# Autodesk Inventor assembly: Final Assembly
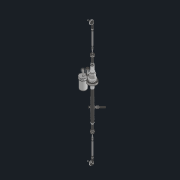
[picture p0: Inventor's stored thumbnail of the model, 180x180]
Saved by Autodesk Inventor 2021 (Build 250183000, 183)
## iProperties
Created: 2020-10-21
Part Number: Final Assembly
Document SubType Name: Assembly
Designer: Tang Kang Ning
Mass: 19906 g
Surface Area: 15225.4 cm^2
Volume: 4263.88 cm^3
Density: 4.66852 g/cm^3
Author: Tang Kang Ning
## Documents named in this file (41)
- C:\Users\teuge\OneDrive - Curtin University of Technology Australia\Y4S2\DFM\Group Project\CAD\Final Assembly.iam
- C:\Users\teuge\OneDrive - Curtin University of Technology Australia\Y4S2\DFM\Group Project\CAD\Parts\Steering Rack.ipt
- C:\Users\teuge\OneDrive - Curtin University of Technology Australia\Y4S2\DFM\Group Project\CAD\Parts\Shell Body.ipt
- C:\Users\teuge\OneDrive - Curtin University of Technology Australia\Y4S2\DFM\Group Project\CAD\Parts\Assemblies\Bearing2.iam
- C:\Users\teuge\OneDrive - Curtin University of Technology Australia\Y4S2\DFM\Group Project\CAD\Parts\Steering Gear.ipt
- C:\Users\teuge\OneDrive - Curtin University of Technology Australia\Y4S2\DFM\Group Project\CAD\Parts\Steering Shaft.ipt
- C:\Users\teuge\OneDrive - Curtin University of Technology Australia\Y4S2\DFM\Group Project\CAD\Parts\Assemblies\Bearing1.iam
- C:\Users\teuge\OneDrive - Curtin University of Technology Australia\Y4S2\DFM\Group Project\CAD\Parts\Assemblies\Motor Assembly.iam
- C:\Users\teuge\OneDrive - Curtin University of Technology Australia\Y4S2\DFM\Group Project\CAD\Parts\Gear Key.ipt
- C:\Users\teuge\OneDrive - Curtin University of Technology Australia\Y4S2\DFM\Group Project\CAD\Parts\Gears\Gear.ipt
- C:\Users\teuge\OneDrive - Curtin University of Technology Australia\Y4S2\DFM\Group Project\CAD\Parts\Intermediate Gear Pin.ipt
- C:\Users\teuge\OneDrive - Curtin University of Technology Australia\Y4S2\DFM\Group Project\CAD\Parts\Assemblies\Bearing7.iam
- C:\Users\teuge\OneDrive - Curtin University of Technology Australia\Y4S2\DFM\Group Project\CAD\Parts\Intermediate Key.ipt
- C:\Users\teuge\OneDrive - Curtin University of Technology Australia\Y4S2\DFM\Group Project\CAD\Parts\Gears\Intermediate.ipt
- C:\Users\teuge\OneDrive - Curtin University of Technology Australia\Y4S2\DFM\Group Project\CAD\Parts\Pinion.ipt
- C:\Users\teuge\OneDrive - Curtin University of Technology Australia\Y4S2\DFM\Group Project\CAD\Parts\PinionMotor Key.ipt
- C:\Users\teuge\OneDrive - Curtin University of Technology Australia\Y4S2\DFM\Group Project\CAD\Parts\Shell Cap.ipt
- C:\Users\teuge\OneDrive - Curtin University of Technology Australia\Y4S2\DFM\Group Project\CAD\Parts\Assemblies\Tie Rod Assembly.iam
- C:\Users\teuge\OneDrive - Curtin University of Technology Australia\Y4S2\DFM\Group Project\CAD\Parts\Screws\ISO 4762 - M6 x 40ISO.ipt
- C:\Users\teuge\OneDrive - Curtin University of Technology Australia\Y4S2\DFM\Group Project\CAD\Parts\Screws\ISO 4762 - M8 x 20ISO.ipt
- C:\Users\teuge\OneDrive - Curtin University of Technology Australia\Y4S2\DFM\Group Project\CAD\Parts\Boot front.ipt
- C:\Users\teuge\OneDrive - Curtin University of Technology Australia\Y4S2\DFM\Group Project\CAD\Parts\Boot Back.ipt
- C:\Users\teuge\OneDrive - Curtin University of Technology Australia\Y4S2\DFM\Group Project\CAD\Final Assembly\Design Accelerator\Involute Spline Connection1.iam
- C:\Users\teuge\OneDrive - Curtin University of Technology Australia\Y4S2\DFM\Group Project\CAD\Final Assembly\Design Accelerator\Bearing1.iam
- C:\Users\teuge\OneDrive - Curtin University of Technology Australia\Y4S2\DFM\Group Project\CAD\Parts\Nut Fastener.ipt
- C:\Users\teuge\OneDrive - Curtin University of Technology Australia\Y4S2\DFM\Group Project\CAD\Parts\Out Tie Rod Joint Cap.ipt
- C:\Users\teuge\OneDrive - Curtin University of Technology Australia\Y4S2\DFM\Group Project\CAD\Parts\Outer Tie Rod Ball.ipt
- C:\Users\teuge\OneDrive - Curtin University of Technology Australia\Y4S2\DFM\Group Project\CAD\Parts\Outer Tie Rod.ipt
- C:\Users\teuge\OneDrive - Curtin University of Technology Australia\Y4S2\DFM\Group Project\CAD\Master\Inner Ball Joint (Body).ipt
- C:\Users\teuge\OneDrive - Curtin University of Technology Australia\Y4S2\DFM\Group Project\CAD\Master\Inner Ball Joint (Cap).ipt
- C:\Users\teuge\OneDrive - Curtin University of Technology Australia\Y4S2\DFM\Group Project\CAD\Master\Tie Rod.ipt
- C:\Users\teuge\OneDrive - Curtin University of Technology Australia\Y4S2\DFM\Group Project\CAD\Master\Ball Screw Nut 1.0.ipt
- C:\Users\teuge\OneDrive - Curtin University of Technology Australia\Y4S2\DFM\Group Project\CAD\Parts\Ball Screw Balls.ipt
- C:\Users\teuge\OneDrive - Curtin University of Technology Australia\Y4S2\DFM\Group Project\CAD\Master\Front Returd Mech.ipt
- C:\Users\teuge\OneDrive - Curtin University of Technology Australia\Y4S2\DFM\Group Project\CAD\Master\BallScrewNut Cap.ipt
- C:\Users\teuge\OneDrive - Curtin University of Technology Australia\Y4S2\DFM\Group Project\CAD\Final Assembly\AIP\FEA\dejyt38kg.fins
- C:\Users\teuge\OneDrive - Curtin University of Technology Australia\Y4S2\DFM\Group Project\CAD\Final Assembly\AIP\FEA\dejyt38kg.fsat
- C:\Users\teuge\OneDrive - Curtin University of Technology Australia\Y4S2\DFM\Group Project\CAD\Final Assembly\AIP\FEA\dejyt38kg.ftes
- C:\Users\teuge\OneDrive - Curtin University of Technology Australia\Y4S2\DFM\Group Project\CAD\Final Assembly\AIP\FEA\dejyt38kg.fwiz
- C:\Users\teuge\OneDrive - Curtin University of Technology Australia\Y4S2\DFM\Group Project\CAD\Final Assembly\AIP\FEA\dekbs9e9s.fmsh
- C:\Users\teuge\OneDrive - Curtin University of Technology Australia\Y4S2\DFM\Group Project\CAD\Final Assembly\AIP\FEA\dekbs9e9t.fres
## Components (51 placed, 31 different names)
1. Steering Rack:1 — Mate:1, Mate:2, Mate:3, Mate:4, Mate:5, Position Adjust, Mate:45, Mate:49, Mate:50, Flush:6, Mate:85, Mate:87, Mate:127, Mate:133, Mate:134
2. Bearing:1 [sub-assembly] — Mate:48
3. Bearing:2 [sub-assembly] — Mate:28
4. Steering Gear:1 — Mate:11, Mate:14
5. Steering Shaft:1 — Mate:11, Mate:12, Flush:1, Mate:13, Mate:14, Position Adjust, Mate:74, Mate:75
6. Bearing:3 [sub-assembly] — Mate:12, Flush:1, Mate:15
7. Motor Assembly:1 [sub-assembly] — Mate:17, Mate:18, Mate:19, Mate:20, Mate:39, Mate:40, Mate:42, Mate:60, Mate:61, Mate:62, Mate:63, Mate:64, Mate:132
8. Gear Key:1 — Mate:79, Mate:125, Mate:126, Mate:129
9. Gear:1 — Flush:4, Mate:79, Mate:128
10. Intermediate Gear Pin:1 — Mate:29, Mate:30, Mate:32, Flush:2, Mate:33, Flush:3, Mate:34, Mate:131
11. Bearing:4 [sub-assembly] — Mate:32, Flush:2, Mate:37, Mate:38
12. Intermediate Key:1 — Mate:29, Mate:30, Mate:35, Mate:36, Mate:131
13. Bearing:5 [sub-assembly] — Mate:33, Flush:3, Mate:130
14. Intermediate:1 — Mate:34, Mate:35, Mate:36, Flush:4, Flush:5
15. Pinion:1 — Mate:42, Mate:43, Mate:44, Flush:5
16. PinionMotor Key:1 — Mate:39, Mate:40, Mate:43, Mate:44, Mate:132
17. Boot front:1 — Mate:70, Mate:71
18. Boot Back:1 — Mate:72, Mate:73
19. Involute Spline Connection:1 [sub-assembly]
20. Bearing:6 [sub-assembly] — Mate:74, Mate:75
21. Out Tie Rod Joint Cap:1 — Mate:102, Mate:103
22. Outer Tie Rod Ball:1 — Mate:82, Mate:101, Mate:112
23. Outer Tie Rod:1 — Mate:82, Mate:101, Mate:102, Mate:103, Mate:104, Mate:110
24. Out Tie Rod Joint Cap:2 — Mate:84, Mate:99
25. Outer Tie Rod Ball:2 — Mate:83, Mate:84, Mate:100, Mate:111
26. Outer Tie Rod:2 — Mate:83, Mate:98, Mate:99, Mate:100, Mate:107
27. Inner Ball Joint (Body):1 — Mate:85, Mate:93, Mate:94, Mate:134
28. Inner Ball Joint (Cap):1 — Mate:93, Mate:94, Mate:95, Mate:97
29. Tie Rod:1 — Mate:95, Mate:97, Mate:98, Mate:105, Mate:106
30. Inner Ball Joint (Body):2 — Mate:87, Mate:90, Mate:91, Mate:92, Mate:133
31. Inner Ball Joint (Cap):2 — Mate:90, Mate:91, Mate:96
32. Tie Rod:2 — Mate:92, Mate:96, Mate:104, Mate:108, Mate:109
33. Nut Fastener:1 — Mate:108, Mate:109, Mate:110
34. Nut Fastener:2 — Mate:105, Mate:106, Mate:107
35. Ball Screw Nut 1.0:1 — Mate:113, Mate:114, Mate:115, Mate:116, Mate:117, Mate:118, Mate:119, Mate:120, Mate:121, Mate:122, Mate:123, Mate:124, Mate:125, Mate:126, Mate:127, Mate:128, Mate:129
36. Ball Screw Balls:1 — Mate:113, Mate:114
37. Front Returd Mech:1 — Mate:115, Mate:116, Mate:117
38. Front Returd Mech:2 — Mate:118, Mate:119, Mate:120
39. BallScrewNut Cap:1 — Mate:122, Mate:123
40. BallScrewNut Cap:2 — Mate:121, Mate:124
41. ISO 4762 - M6 x 40ISO:1 — Mate:60, Mate:63
42. ISO 4762 - M8 x 20ISO:1 — Mate:57, Mate:65
43. ISO 4762 - M6 x 40ISO:2 — Mate:61, Mate:64
44. ISO 4762 - M8 x 20ISO:2 — Mate:56, Mate:66
45. ISO 4762 - M6 x 40ISO:3 — Mate:59, Mate:62
46. ISO 4762 - M8 x 20ISO:3 — Mate:58, Mate:67
47. ISO 4762 - M8 x 20ISO:4 — Mate:55, Mate:68
48. Shell Body:1 — Mate:1, Mate:2, Mate:13, Mate:15, Mate:17, Mate:18, Mate:19, Mate:20, Mate:28, Mate:37, Mate:38, Mate:46, Mate:47, Mate:56, Mate:59, Mate:72, Mate:73
49. Shell Cap:1 — Mate:45, Mate:46, Mate:47, Mate:48, Mate:55, Mate:57, Mate:58, Mate:65, Mate:66, Mate:67, Mate:68, Mate:71, Mate:130
50. Tie Rod Assembly:1 [sub-assembly] — Mate:50, Mate:54, Mate:70
51. Tie Rod Assembly:2 [sub-assembly] — Mate:49, Mate:53
## Relationships (115: Mate 109, Flush 6)
- Mate:1: Steering Rack:1 ↔ Shell Body:1
- Mate:2: Steering Rack:1 ↔ Shell Body:1
- Mate:3: Steering Rack:1
- Mate:4: Steering Rack:1
- Mate:5: Steering Rack:1
- Mate:11: Steering Gear:1 ↔ Steering Shaft:1
- Mate:12: Steering Shaft:1 ↔ Bearing:3
- Flush:1: Steering Shaft:1 ↔ Bearing:3
- Mate:13: Steering Shaft:1 ↔ Shell Body:1
- Mate:14: Steering Gear:1 ↔ Steering Shaft:1
- Mate:15: Bearing:3 ↔ Shell Body:1
- Position Adjust [Mate] (-2.75 mm): Steering Rack:1 ↔ Steering Shaft:1
- Mate:17: Motor Assembly:1 ↔ Shell Body:1
- Mate:18: Motor Assembly:1 ↔ Shell Body:1
- Mate:19: Motor Assembly:1 ↔ Shell Body:1
- Mate:20: Motor Assembly:1 ↔ Shell Body:1
- Mate:28: Bearing:2 ↔ Shell Body:1
- Mate:29: Intermediate Gear Pin:1 ↔ Intermediate Key:1
- Mate:30: Intermediate Gear Pin:1 ↔ Intermediate Key:1
- Mate:32: Intermediate Gear Pin:1 ↔ Bearing:4
- Flush:2: Intermediate Gear Pin:1 ↔ Bearing:4
- Mate:33: Intermediate Gear Pin:1 ↔ Bearing:5
- Flush:3: Intermediate Gear Pin:1 ↔ Bearing:5
- Mate:34: Intermediate Gear Pin:1 ↔ Intermediate:1
- Mate:35: Intermediate Key:1 ↔ Intermediate:1
- Mate:36: Intermediate Key:1 ↔ Intermediate:1
- Mate:37: Bearing:4 ↔ Shell Body:1
- Mate:38: Bearing:4 ↔ Shell Body:1
- Flush:4: Gear:1 ↔ Intermediate:1
- Mate:39: Motor Assembly:1 ↔ PinionMotor Key:1
- Mate:40: Motor Assembly:1 ↔ PinionMotor Key:1
- Mate:42: Motor Assembly:1 ↔ Pinion:1
- Mate:43: Pinion:1 ↔ PinionMotor Key:1
- Mate:44: Pinion:1 ↔ PinionMotor Key:1
- Flush:5: Intermediate:1 ↔ Pinion:1
- Mate:45: Steering Rack:1 ↔ Shell Cap:1
- Mate:46: Shell Body:1 ↔ Shell Cap:1
- Mate:47: Shell Body:1 ↔ Shell Cap:1
- Mate:48: Bearing:1 ↔ Shell Cap:1
- Mate:49: Steering Rack:1 ↔ Tie Rod Assembly:2
- Mate:50: Steering Rack:1 ↔ Tie Rod Assembly:1
- Mate:53: Tie Rod Assembly:2
- Mate:54: Tie Rod Assembly:1
- Mate:55: ISO 4762 - M8 x 20ISO:4 ↔ Shell Cap:1
- Mate:56: ISO 4762 - M8 x 20ISO:2 ↔ Shell Body:1
- Mate:57: ISO 4762 - M8 x 20ISO:1 ↔ Shell Cap:1
- Mate:58: ISO 4762 - M8 x 20ISO:3 ↔ Shell Cap:1
- Mate:59: ISO 4762 - M6 x 40ISO:3 ↔ Shell Body:1
- Mate:60: Motor Assembly:1 ↔ ISO 4762 - M6 x 40ISO:1
- Mate:61: Motor Assembly:1 ↔ ISO 4762 - M6 x 40ISO:2
- Mate:62: Motor Assembly:1 ↔ ISO 4762 - M6 x 40ISO:3
- Mate:63: Motor Assembly:1 ↔ ISO 4762 - M6 x 40ISO:1
- Mate:64: Motor Assembly:1 ↔ ISO 4762 - M6 x 40ISO:2
- Mate:65: ISO 4762 - M8 x 20ISO:1 ↔ Shell Cap:1
- Mate:66: ISO 4762 - M8 x 20ISO:2 ↔ Shell Cap:1
- Mate:67: ISO 4762 - M8 x 20ISO:3 ↔ Shell Cap:1
- Mate:68: ISO 4762 - M8 x 20ISO:4 ↔ Shell Cap:1
- Flush:6: Steering Rack:1
- Mate:70: Boot front:1 ↔ Tie Rod Assembly:1
- Mate:71: Boot front:1 ↔ Shell Cap:1
- Mate:72: Boot Back:1 ↔ Shell Body:1
- Mate:73: Boot Back:1 ↔ Shell Body:1
- Mate:74: Steering Shaft:1 ↔ Bearing:6
- Mate:75: Steering Shaft:1 ↔ Bearing:6
- Mate:79: Gear Key:1 ↔ Gear:1
- Mate:82: Outer Tie Rod Ball:1 ↔ Outer Tie Rod:1
- Mate:83: Outer Tie Rod Ball:2 ↔ Outer Tie Rod:2
- Mate:84: Out Tie Rod Joint Cap:2 ↔ Outer Tie Rod Ball:2
- Mate:85: Steering Rack:1 ↔ Inner Ball Joint (Body):1
- Mate:87: Steering Rack:1 ↔ Inner Ball Joint (Body):2
- Mate:90: Inner Ball Joint (Body):2 ↔ Inner Ball Joint (Cap):2
- Mate:91: Inner Ball Joint (Body):2 ↔ Inner Ball Joint (Cap):2
- Mate:92: Inner Ball Joint (Body):2 ↔ Tie Rod:2
- Mate:93: Inner Ball Joint (Body):1 ↔ Inner Ball Joint (Cap):1
- Mate:94: Inner Ball Joint (Body):1 ↔ Inner Ball Joint (Cap):1
- Mate:95: Inner Ball Joint (Cap):1 ↔ Tie Rod:1
- Mate:96: Inner Ball Joint (Cap):2 ↔ Tie Rod:2
- Mate:97: Inner Ball Joint (Cap):1 ↔ Tie Rod:1
- Mate:98: Outer Tie Rod:2 ↔ Tie Rod:1
- Mate:99: Out Tie Rod Joint Cap:2 ↔ Outer Tie Rod:2
- Mate:100: Outer Tie Rod Ball:2 ↔ Outer Tie Rod:2
- Mate:101: Outer Tie Rod Ball:1 ↔ Outer Tie Rod:1
- Mate:102: Out Tie Rod Joint Cap:1 ↔ Outer Tie Rod:1
- Mate:103: Out Tie Rod Joint Cap:1 ↔ Outer Tie Rod:1
- Mate:104: Outer Tie Rod:1 ↔ Tie Rod:2
- Mate:105: Tie Rod:1 ↔ Nut Fastener:2
- Mate:106 (7.8 mm): Tie Rod:1 ↔ Nut Fastener:2
- Mate:107: Outer Tie Rod:2 ↔ Nut Fastener:2
- Mate:108: Tie Rod:2 ↔ Nut Fastener:1
- Mate:109 (7.8 mm): Tie Rod:2 ↔ Nut Fastener:1
- Mate:110: Outer Tie Rod:1 ↔ Nut Fastener:1
- Mate:111: Outer Tie Rod Ball:2
- Mate:112: Outer Tie Rod Ball:1
- Mate:113: Ball Screw Nut 1.0:1 ↔ Ball Screw Balls:1
- Mate:114: Ball Screw Nut 1.0:1 ↔ Ball Screw Balls:1
- Mate:115: Ball Screw Nut 1.0:1 ↔ Front Returd Mech:1
- Mate:116: Ball Screw Nut 1.0:1 ↔ Front Returd Mech:1
- Mate:117: Ball Screw Nut 1.0:1 ↔ Front Returd Mech:1
- Mate:118: Ball Screw Nut 1.0:1 ↔ Front Returd Mech:2
- Mate:119: Ball Screw Nut 1.0:1 ↔ Front Returd Mech:2
- Mate:120: Ball Screw Nut 1.0:1 ↔ Front Returd Mech:2
- Mate:121: Ball Screw Nut 1.0:1 ↔ BallScrewNut Cap:2
- Mate:122: Ball Screw Nut 1.0:1 ↔ BallScrewNut Cap:1
- Mate:123: Ball Screw Nut 1.0:1 ↔ BallScrewNut Cap:1
- Mate:124: Ball Screw Nut 1.0:1 ↔ BallScrewNut Cap:2
- Mate:125: Gear Key:1 ↔ Ball Screw Nut 1.0:1
- Mate:126: Gear Key:1 ↔ Ball Screw Nut 1.0:1
- Mate:127: Steering Rack:1 ↔ Ball Screw Nut 1.0:1
- Mate:128: Gear:1 ↔ Ball Screw Nut 1.0:1
- Mate:129: Gear Key:1 ↔ Ball Screw Nut 1.0:1
- Mate:130: Bearing:5 ↔ Shell Cap:1
- Mate:131: Intermediate Gear Pin:1 ↔ Intermediate Key:1
- Mate:132: Motor Assembly:1 ↔ PinionMotor Key:1
- Mate:133: Steering Rack:1 ↔ Inner Ball Joint (Body):2
- Mate:134: Steering Rack:1 ↔ Inner Ball Joint (Body):1
## Named parameters: FrontBootLength = 153.75 mm, BackBootLength = 159.25 mm, sa_1 = 5000, sa_0 = 1e+07, sa_eq_min = 8.4868, sa_eq_max = 86440.6, sa_d_min = 0 mm, sa_d_max = 0.00033 mm, sa_sf_min = 15, sa_sf_max = 15, sa_ps1_min = -15819.8, sa_ps1_max = 74936.7, sa_ps3_min = -46327, sa_ps3_max = 6980.51, sa_eqst_min = 7e-08, sa_eqst_max = 3.88e-05, sa_st1_min = -8.67e-05, sa_st1_max = 4.138e-05, sa_st3_min = -3.208e-05, sa_st3_max = 9.918e-05, sa_cp_min = 0.0488, sa_cp_max = 157189, sa_2 = 100000, sa_3 = 100000, sa_4 = 100000
note: some values were not read from the file. Shown as the stored number, unit unknown: "sa_1", "sa_0", "sa_eq_min", "sa_eq_max", "sa_ps1_min", "sa_ps1_max", "sa_ps3_min", "sa_ps3_max", "sa_cp_min", "sa_cp_max", "sa_2", "sa_3", "sa_4".
